# Autodesk Inventor assembly: CE-9.3.2
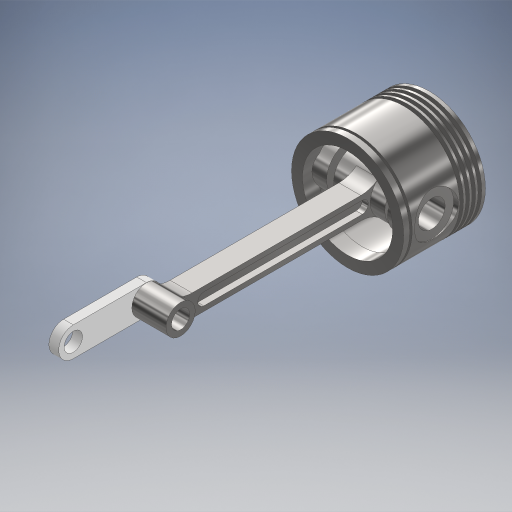
[picture p0: Inventor's stored thumbnail of the model, 512x512]
Saved by Autodesk Inventor 2024 (Build 280153000, 153)
## iProperties
Created: 2024-03-22
Part Number: CE-9.3.2
Document SubType Name: Assembly
Designer: Alex
Author: Alex
## Documents named in this file (4)
- C:\Shared\alex-bartella-schoolwork\4z03\Week 10\CE-9.3.2.iam
- C:\Shared\alex-bartella-schoolwork\4z03\Week 10\CE-9.3.2-crank.ipt
- C:\Shared\alex-bartella-schoolwork\4z03\Week 10\arm and piston\Arm.ipt
- C:\Shared\alex-bartella-schoolwork\4z03\Week 10\arm and piston\Piston.ipt
## Components (3 placed, 3 different names)
1. CE-9.3.2-crank:1 — Mate:1, Flush:1, Cylindrical:1, Mate:2
2. Arm:1 — Cylindrical:1, Mate:2, Mate:3, Mate:4
3. Piston:1 — Mate:3, Mate:4, Flush:6
## Relationships (7: Mate 4, Flush 2, CylindricalJoint 1)
- Mate:1: CE-9.3.2-crank:1
- Flush:1: CE-9.3.2-crank:1
- Cylindrical:1: CE-9.3.2-crank:1 ↔ Arm:1
- Mate:2: CE-9.3.2-crank:1 ↔ Arm:1
- Mate:3: Arm:1 ↔ Piston:1
- Mate:4 (4 mm): Arm:1 ↔ Piston:1
- Flush:6: Piston:1
## Named parameters: Simulation_Timeline = 0
